# Autodesk Inventor assembly: 2mm_cnc_v1
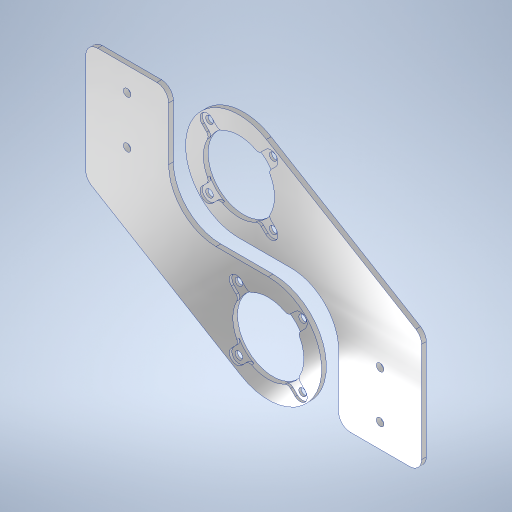
[picture p0: Inventor's stored thumbnail of the model, 512x512]
Saved by Autodesk Inventor 2024.3 (Build 283343010, 343A)
## iProperties
Created: 2025-07-12
Part Number: 2mm_cnc_v1
Document SubType Name: Assembly
Designer: tanoue_kota
Author: tanoue_kota
## Documents named in this file (2)
- C:\Users\kshau\Documents\inventor\Create_ViperX\Create_ViperX_ALOHA\FlatPattern\2mm_cnc_v1.iam
- C:\Users\kshau\Documents\inventor\Create_ViperX\Create_ViperX_ALOHA\UpperArm_Component_v2\upperarm_fixplate2_forR0.ipt
## Components (2 placed, 1 different names)
1. upperarm_fixplate2_forR0:1 — フラッシュ:1, メイト:1
2. upperarm_fixplate2_forR0:2 — フラッシュ:1, メイト:1
## Relationships (2: Flush 1, Mate 1)
- フラッシュ:1 [Flush]: upperarm_fixplate2_forR0:1 ↔ upperarm_fixplate2_forR0:2
- メイト:1 [Mate] (8 mm): upperarm_fixplate2_forR0:1 ↔ upperarm_fixplate2_forR0:2
